# Autodesk Inventor assembly: airhockeybot_x_traverse_sumulation
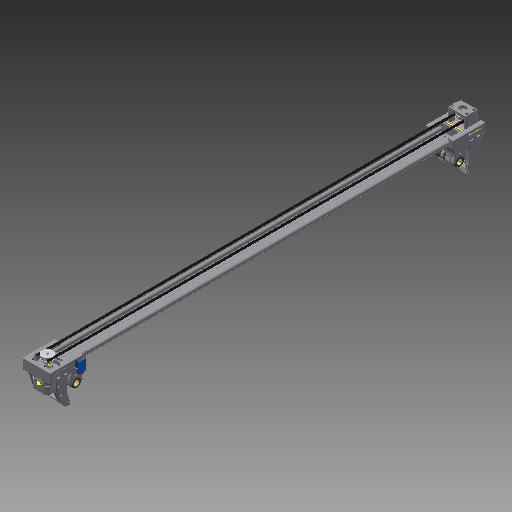
[picture p0: Inventor's stored thumbnail of the model, 512x512]
Saved by Autodesk Inventor 2019.3 (Build 233278000, 278)
## iProperties
Created: 2020-08-23
Part Number: airhockeybot_x_traverse_sumulation
Material: Generisch
Document SubType Name: Assembly
Designer: Nicolas Frick
Author: Nicolas Frick
## Documents named in this file (17)
- C:\Users\Nicolas Frick\Sync\OneDrive\airhockeybot\mechanical_design\common_cad_parts\sim_models\airhockeybot_x_traverse_sumulation.iam
- C:\Users\Nicolas Frick\Sync\OneDrive\airhockeybot\mechanical_design\inventor\Pulley.iam
- C:\Users\Nicolas Frick\Sync\OneDrive\airhockeybot\mechanical_design\inventor\igus\RJUM_01_12_3.ipt
- C:\Users\Nicolas Frick\Sync\OneDrive\airhockeybot\mechanical_design\inventor\Switch CMV101D\CNDT_CMV101D.ipt
- C:\Users\Nicolas Frick\Sync\OneDrive\airhockeybot\mechanical_design\inventor\Nema 17HS5425\Assembly1.iam
- C:\Users\Nicolas Frick\Sync\OneDrive\airhockeybot\mechanical_design\inventor\GT2 40T 5mm Bore 6mm wide pulley\GT2 40T 5 Bore v2.iam
- C:\Users\Nicolas Frick\Sync\OneDrive\airhockeybot\mechanical_design\inventor\igus\WS_10_40_200_2_modify.ipt
- C:\Users\Nicolas Frick\Sync\OneDrive\airhockeybot\mechanical_design\inventor\GT2 Belt 6mm\GT2 Belt 6mm x 40mm.ipt
- C:\Users\Nicolas Frick\Sync\OneDrive\airhockeybot\mechanical_design\inventor\Upper_left_fixture.ipt
- C:\Users\Nicolas Frick\Sync\OneDrive\airhockeybot\mechanical_design\inventor\Belt_clamp.ipt
- C:\Users\Nicolas Frick\Sync\OneDrive\airhockeybot\mechanical_design\inventor\Belt_clamp_mirrored.ipt
- C:\Users\Nicolas Frick\Sync\OneDrive\airhockeybot\mechanical_design\inventor\Distance_lin.ipt
- C:\Users\Nicolas Frick\Sync\OneDrive\airhockeybot\mechanical_design\inventor\Upper_right_fixture.ipt
- C:\Users\Nicolas Frick\Sync\OneDrive\airhockeybot\mechanical_design\inventor\Upper_bearing_support_inside.ipt
- C:\Users\Nicolas Frick\Sync\OneDrive\airhockeybot\mechanical_design\inventor\Upper_bearing_support_outside.ipt
- C:\Users\Nicolas Frick\Sync\OneDrive\airhockeybot\mechanical_design\inventor\Stiff_motor.ipt
- C:\Users\Nicolas Frick\Sync\OneDrive\airhockeybot\mechanical_design\inventor\Stiff.ipt
## Components (73 placed, 16 different names)
1. RJUM_01_12_3:1 — Passend:108, Fluchtend:37, Passend:115
2. RJUM_01_12_3:2 — Passend:107, Fluchtend:36
3. WS_10_40_200_2_modify:1 — Passend:187, Passend:188, Passend:189
4. RJUM_01_12_3:3 — Passend:118, Passend:121, Fluchtend:45
5. RJUM_01_12_3:4 — Passend:119, Passend:122
6. Upper_left_fixture:1 — Passend:107, Passend:108, Fluchtend:36, Fluchtend:37, Fluchtend:38, Fluchtend:39, Fluchtend:40, Fluchtend:44, Passend:146, Passend:147, Passend:187, Passend:189, Passend:191, Fluchtend:75, Fluchtend:76
7. Assembly1:3 [sub-assembly] — Passend:105, Passend:106, Fluchtend:38, Fluchtend:39, Fluchtend:40
8. GT2 40T 5 Bore v2:3 [sub-assembly] — Passend:105, Passend:106
9. Belt_clamp:1 — Fluchtend:41, Fluchtend:42, Passend:147, Passend:195, Passend:197, Passend:198
10. Belt_clamp_mirrored:1 — Fluchtend:41, Fluchtend:42, Passend:146
11. Distance_lin:1 — Passend:115
12. Upper_right_fixture:1 — Fluchtend:44, Passend:118, Passend:119, Fluchtend:45, Passend:131, Passend:132, Passend:144, Passend:145, Passend:188
13. Distance_lin:2 — Passend:121, Passend:122
14. Upper_bearing_support_inside:1 — Passend:127, Passend:128, Fluchtend:48, Fluchtend:49, Passend:130, Passend:131, Passend:132
15. Pulley:3 [sub-assembly] — Passend:127, Passend:128, Passend:129
16. Upper_bearing_support_outside:1 — Fluchtend:48, Fluchtend:49, Passend:129, Passend:130, Passend:140, Passend:141, Fluchtend:52, Passend:142, Passend:143, Fluchtend:53
17. Belt_clamp:2 — Fluchtend:50, Fluchtend:51, Passend:144, Passend:206, Passend:208
18. Belt_clamp_mirrored:2 — Fluchtend:50, Fluchtend:51, Passend:145, Passend:207
19. CNDT_CMV101D:6 — Passend:191, Fluchtend:75, Fluchtend:76
20. Stiff_motor:1 — Passend:195, Passend:197, Passend:198
21. Stiff:1 — Passend:206, Passend:207, Passend:208
22. GT2 Belt 6mm x 40mm:98 — Passend:140, Passend:141, Fluchtend:52
23. GT2 Belt 6mm x 40mm:99
24. GT2 Belt 6mm x 40mm:100
25. GT2 Belt 6mm x 40mm:101
26. GT2 Belt 6mm x 40mm:102
27. GT2 Belt 6mm x 40mm:103
28. GT2 Belt 6mm x 40mm:104
29. GT2 Belt 6mm x 40mm:105
30. GT2 Belt 6mm x 40mm:106
31. GT2 Belt 6mm x 40mm:107
32. GT2 Belt 6mm x 40mm:108
33. GT2 Belt 6mm x 40mm:109
34. GT2 Belt 6mm x 40mm:110
35. GT2 Belt 6mm x 40mm:111
36. GT2 Belt 6mm x 40mm:112
37. GT2 Belt 6mm x 40mm:113
38. GT2 Belt 6mm x 40mm:114
39. GT2 Belt 6mm x 40mm:115
40. GT2 Belt 6mm x 40mm:116
41. GT2 Belt 6mm x 40mm:117
42. GT2 Belt 6mm x 40mm:118
43. GT2 Belt 6mm x 40mm:119
44. GT2 Belt 6mm x 40mm:120
45. GT2 Belt 6mm x 40mm:121
46. GT2 Belt 6mm x 40mm:122
47. GT2 Belt 6mm x 40mm:123
48. GT2 Belt 6mm x 40mm:97 — Passend:142, Passend:143, Fluchtend:53
49. GT2 Belt 6mm x 40mm:124
50. GT2 Belt 6mm x 40mm:125
51. GT2 Belt 6mm x 40mm:126
52. GT2 Belt 6mm x 40mm:127
53. GT2 Belt 6mm x 40mm:128
54. GT2 Belt 6mm x 40mm:129
55. GT2 Belt 6mm x 40mm:130
56. GT2 Belt 6mm x 40mm:131
57. GT2 Belt 6mm x 40mm:132
58. GT2 Belt 6mm x 40mm:133
59. GT2 Belt 6mm x 40mm:134
60. GT2 Belt 6mm x 40mm:135
61. GT2 Belt 6mm x 40mm:136
62. GT2 Belt 6mm x 40mm:137
63. GT2 Belt 6mm x 40mm:138
64. GT2 Belt 6mm x 40mm:139
65. GT2 Belt 6mm x 40mm:140
66. GT2 Belt 6mm x 40mm:141
67. GT2 Belt 6mm x 40mm:142
68. GT2 Belt 6mm x 40mm:143
69. GT2 Belt 6mm x 40mm:144
70. GT2 Belt 6mm x 40mm:145
71. GT2 Belt 6mm x 40mm:146
72. GT2 Belt 6mm x 40mm:147
73. GT2 Belt 6mm x 40mm:148
## Component patterns: (26 elements, first: GT2 Belt 6mm x 40mm:98), (26 elements, first: GT2 Belt 6mm x 40mm:97)
## Relationships (50: Mate 33, Flush 17)
- Passend:105 [Mate]: Assembly1:3 ↔ GT2 40T 5 Bore v2:3
- Passend:106 [Mate] (1.3 mm): Assembly1:3 ↔ GT2 40T 5 Bore v2:3
- Passend:107 [Mate]: RJUM_01_12_3:2 ↔ Upper_left_fixture:1
- Passend:108 [Mate]: RJUM_01_12_3:1 ↔ Upper_left_fixture:1
- Fluchtend:36 [Flush]: RJUM_01_12_3:2 ↔ Upper_left_fixture:1
- Fluchtend:37 [Flush]: RJUM_01_12_3:1 ↔ Upper_left_fixture:1
- Fluchtend:38 [Flush] (13 mm): Upper_left_fixture:1 ↔ Assembly1:3
- Fluchtend:39 [Flush] (5 mm): Upper_left_fixture:1 ↔ Assembly1:3
- Fluchtend:40 [Flush] (10 mm): Upper_left_fixture:1 ↔ Assembly1:3
- Fluchtend:41 [Flush]: Belt_clamp:1 ↔ Belt_clamp_mirrored:1
- Fluchtend:42 [Flush]: Belt_clamp:1 ↔ Belt_clamp_mirrored:1
- Passend:115 [Mate]: RJUM_01_12_3:1 ↔ Distance_lin:1
- Fluchtend:44 [Flush]: Upper_left_fixture:1 ↔ Upper_right_fixture:1
- Passend:118 [Mate]: RJUM_01_12_3:3 ↔ Upper_right_fixture:1
- Passend:119 [Mate]: RJUM_01_12_3:4 ↔ Upper_right_fixture:1
- Passend:121 [Mate]: RJUM_01_12_3:3 ↔ Distance_lin:2
- Passend:122 [Mate]: RJUM_01_12_3:4 ↔ Distance_lin:2
- Fluchtend:45 [Flush]: RJUM_01_12_3:3 ↔ Upper_right_fixture:1
- Passend:127 [Mate]: Upper_bearing_support_inside:1 ↔ Pulley:3
- Passend:128 [Mate]: Upper_bearing_support_inside:1 ↔ Pulley:3
- Fluchtend:48 [Flush]: Upper_bearing_support_inside:1 ↔ Upper_bearing_support_outside:1
- Fluchtend:49 [Flush]: Upper_bearing_support_inside:1 ↔ Upper_bearing_support_outside:1
- Passend:129 [Mate]: Pulley:3 ↔ Upper_bearing_support_outside:1
- Passend:130 [Mate]: Upper_bearing_support_inside:1 ↔ Upper_bearing_support_outside:1
- Passend:131 [Mate] (0.1 mm): Upper_right_fixture:1 ↔ Upper_bearing_support_inside:1
- Passend:132 [Mate]: Upper_right_fixture:1 ↔ Upper_bearing_support_inside:1
- Fluchtend:50 [Flush]: Belt_clamp:2 ↔ Belt_clamp_mirrored:2
- Fluchtend:51 [Flush]: Belt_clamp:2 ↔ Belt_clamp_mirrored:2
- Passend:140 [Mate] (2.5 mm): Upper_bearing_support_outside:1 ↔ GT2 Belt 6mm x 40mm:98
- Passend:141 [Mate] (5.4 mm): Upper_bearing_support_outside:1 ↔ GT2 Belt 6mm x 40mm:98
- Fluchtend:52 [Flush] (20 mm): Upper_bearing_support_outside:1 ↔ GT2 Belt 6mm x 40mm:98
- Passend:142 [Mate] (2.5 mm): Upper_bearing_support_outside:1 ↔ GT2 Belt 6mm x 40mm:97
- Passend:143 [Mate] (5.5 mm): Upper_bearing_support_outside:1 ↔ GT2 Belt 6mm x 40mm:97
- Fluchtend:53 [Flush] (20 mm): Upper_bearing_support_outside:1 ↔ GT2 Belt 6mm x 40mm:97
- Passend:144 [Mate]: Upper_right_fixture:1 ↔ Belt_clamp:2
- Passend:145 [Mate]: Upper_right_fixture:1 ↔ Belt_clamp_mirrored:2
- Passend:146 [Mate]: Upper_left_fixture:1 ↔ Belt_clamp_mirrored:1
- Passend:147 [Mate]: Upper_left_fixture:1 ↔ Belt_clamp:1
- Passend:187 [Mate]: WS_10_40_200_2_modify:1 ↔ Upper_left_fixture:1
- Passend:188 [Mate]: WS_10_40_200_2_modify:1 ↔ Upper_right_fixture:1
- Passend:189 [Mate]: WS_10_40_200_2_modify:1 ↔ Upper_left_fixture:1
- Passend:191 [Mate]: Upper_left_fixture:1 ↔ CNDT_CMV101D:6
- Fluchtend:75 [Flush] (1 mm): Upper_left_fixture:1 ↔ CNDT_CMV101D:6
- Fluchtend:76 [Flush] (4 mm): Upper_left_fixture:1 ↔ CNDT_CMV101D:6
- Passend:195 [Mate]: Belt_clamp:1 ↔ Stiff_motor:1
- Passend:197 [Mate]: Belt_clamp:1 ↔ Stiff_motor:1
- Passend:198 [Mate]: Belt_clamp:1 ↔ Stiff_motor:1
- Passend:206 [Mate]: Belt_clamp:2 ↔ Stiff:1
- Passend:207 [Mate]: Belt_clamp_mirrored:2 ↔ Stiff:1
- Passend:208 [Mate]: Belt_clamp:2 ↔ Stiff:1
